# Autodesk Inventor assembly: Drifter_Assembly
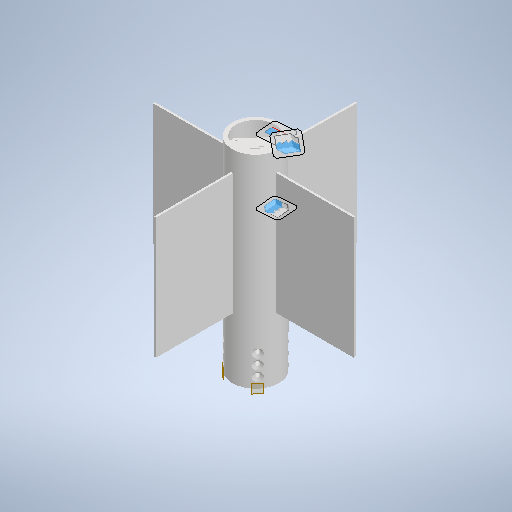
[picture p0: Inventor's stored thumbnail of the model, 512x512]
Saved by Autodesk Inventor 2025 (Build 290162000, 162)
## iProperties
Created: 2024-05-17
Part Number: Drifter_Assembly
Document SubType Name: Assembly
Designer: sml6042
Author: sml6042
## Documents named in this file (5)
- C:\Users\caa9947\Desktop\smartcoastCAD\body\Drifter_Assembly.iam
- C:\Users\caa9947\Desktop\smartcoastCAD\body\Drifter_Body.ipt
- C:\Users\sml6042\Downloads\85065K33_Chemical-Resistant PVC U-Channel\85065K33_Chemical-Resistant PVC U-Channel.ipt
- C:\Users\caa9947\Desktop\smartcoastCAD\body\Drag_Vane.ipt
- C:\Users\caa9947\Downloads\Chassis_Assembly (2).iam
## Components (10 placed, 4 different names)
1. Drifter_Body:1 — Mate:1, Flush:1, Tangent:1, Mate:2, Flush:2, Tangent:2, Flush:3, Flush:4, Rotational:1
2. 85065K33_Chemical-Resistant PVC U-Channel:1 — Flush:2, Tangent:2
3. 85065K33_Chemical-Resistant PVC U-Channel:2
4. 85065K33_Chemical-Resistant PVC U-Channel:3 — Rigid:2, Rigid:3
5. 85065K33_Chemical-Resistant PVC U-Channel:4 — Mate:1, Flush:1, Tangent:1
6. Drag_Vane:1
7. Drag_Vane:2 — Rigid:2, Rigid:3, Flush:4
8. Drag_Vane:3
9. Drag_Vane:4 — Flush:3
10. Chassis_Assembly (2):1 [sub-assembly] — Rotational:1
## Relationships (11: Flush 4, Mate 2, Tangent 2, WeldJoint 2, RevoluteJoint 1)
- Mate:1 (100 mm): Drifter_Body:1 ↔ 85065K33_Chemical-Resistant PVC U-Channel:4
- Flush:1 (85 mm): Drifter_Body:1 ↔ 85065K33_Chemical-Resistant PVC U-Channel:4
- Tangent:1: Drifter_Body:1 ↔ 85065K33_Chemical-Resistant PVC U-Channel:4
- Mate:2: Drifter_Body:1
- Flush:2 (85 mm): Drifter_Body:1 ↔ 85065K33_Chemical-Resistant PVC U-Channel:1
- Tangent:2: Drifter_Body:1 ↔ 85065K33_Chemical-Resistant PVC U-Channel:1
- Rigid:2 [WeldJoint]: 85065K33_Chemical-Resistant PVC U-Channel:3 ↔ Drag_Vane:2
- Flush:3 (150 mm): Drifter_Body:1 ↔ Drag_Vane:4
- Rigid:3 [WeldJoint]: 85065K33_Chemical-Resistant PVC U-Channel:3 ↔ Drag_Vane:2
- Flush:4 (150 mm): Drifter_Body:1 ↔ Drag_Vane:2
- Rotational:1 [RevoluteJoint]: Drifter_Body:1 ↔ Chassis_Assembly (2):1
